# Autodesk Inventor assembly: bearings
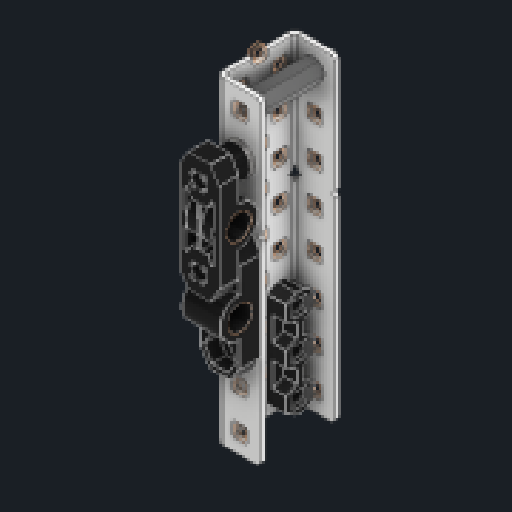
[picture p0: Inventor's stored thumbnail of the model, 512x512]
Saved by Autodesk Inventor 2024 (Build 280153000, 153)
## iProperties
Created: 2023-08-16
Part Number: bearings
Document SubType Name: Assembly
Designer: avere
Author: avere
## Documents named in this file (13)
- D:\vex_robotics\hardware\cad\scrap_v0.1\catapult\bearings.iam
- D:\vex_robotics\hardware\cad\VEX-CAD-Inventor-1.41\Motion\Shaft LS\Bearing Flat Low Profile.ipt
- D:\vex_robotics\hardware\cad\VEX-CAD-Inventor-1.41\Motion\Shaft HS\HS Pillow Bearing Block.ipt
- D:\vex_robotics\hardware\cad\scrap_v0.1\catapult\mirrored_parts\HS Pillow Bearing Block_MIR.ipt
- D:\vex_robotics\hardware\cad\VEX-CAD-Inventor-1.41\Structure\Hardware\Nut Nylon\Nut Nylon - White.ipt
- D:\vex_robotics\hardware\cad\VEX-CAD-Inventor-1.41\Structure\Hardware\Nut Nylon.ipt
- D:\vex_robotics\hardware\cad\VEX-CAD-Inventor-1.41\Motion\Spacers\Spacer Nylon .375 OD\NSpacer .375 OD x .250.ipt
- D:\vex_robotics\hardware\cad\VEX-CAD-Inventor-1.41\Motion\Spacers\Spacer Nylon .375 OD.ipt
- D:\vex_robotics\hardware\cad\VEX-CAD-Inventor-1.41\Motion\Spacers\Washer Steel\SWasher .375 OD x .062500.ipt
- D:\vex_robotics\hardware\cad\VEX-CAD-Inventor-1.41\Motion\Spacers\Washer Steel.ipt
- D:\vex_robotics\hardware\cad\VEX-CAD-Inventor-1.41\Structure\C Channel\Aluminum 1x2x1\Alu C 1x2x1x8.ipt
- D:\vex_robotics\hardware\cad\VEX-CAD-Inventor-1.41\Structure\Standoff\Standoff .875.ipt
- D:\vex_robotics\hardware\cad\VEX-CAD-Inventor-1.41\Structure\Standoff.ipt
## Components (8 placed, 8 different names)
1. Bearing Flat Low Profile:1 — Insert:7, Mate:4
2. HS Pillow Bearing Block:1 — Mate:3, Insert:8, Mate:5
3. HS Pillow Bearing Block_MIR:1 — Mate:3
4. Nut Nylon - White:1
5. NSpacer .375 OD x .250:1 — Insert:6
6. SWasher .375 OD x .062500:1 — Insert:6, Mate:6
7. Alu C 1x2x1x8:1 — Insert:7, Mate:4, Insert:8, Mate:5, Mate:6, Insert:9
8. Standoff .875:1 — Insert:9
## Relationships (10: Insert 6, Mate 4)
- [Insert]: HS Pillow Bearing Block_MIR:1 ↔ Nut Nylon - White:1
- [Insert]: Nut Nylon - White:1 ↔ NSpacer .375 OD x .250:1
- Insert:6: NSpacer .375 OD x .250:1 ↔ SWasher .375 OD x .062500:1
- Mate:3: HS Pillow Bearing Block:1 ↔ HS Pillow Bearing Block_MIR:1
- Insert:7: Bearing Flat Low Profile:1 ↔ Alu C 1x2x1x8:1
- Mate:4: Bearing Flat Low Profile:1 ↔ Alu C 1x2x1x8:1
- Insert:8: HS Pillow Bearing Block:1 ↔ Alu C 1x2x1x8:1
- Mate:5: HS Pillow Bearing Block:1 ↔ Alu C 1x2x1x8:1
- Mate:6: SWasher .375 OD x .062500:1 ↔ Alu C 1x2x1x8:1
- Insert:9: Alu C 1x2x1x8:1 ↔ Standoff .875:1
